# Autodesk Inventor assembly: BATTERY ASSEMBLY
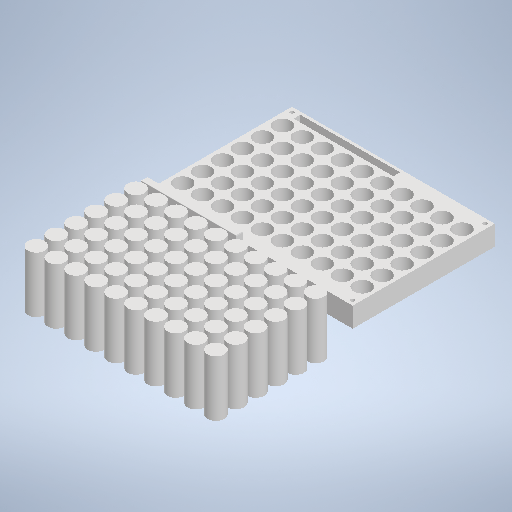
[picture p0: Inventor's stored thumbnail of the model, 512x512]
Saved by Autodesk Inventor 2025.2 (Build 292293000, 293)
## iProperties
Created: 2025-03-22
Part Number: BATTERY ASSEMBLY
Document SubType Name: Assembly
Designer: Mathias
Author: Mathias
## Documents named in this file (4)
- C:\Users\Mathias\Desktop\Projekt Olkassa\Autodesk-inventor-filesharing\BATTERY ASSEMBLY.iam
- C:\Users\Mathias\Desktop\Projekt Olkassa\Autodesk-inventor-filesharing\21700.ipt
- C:\Users\Mathias\Desktop\Projekt Olkassa\Autodesk-inventor-filesharing\BMS.ipt
- C:\Users\Mathias\Desktop\Projekt Olkassa\Autodesk-inventor-filesharing\Battery Holder pt1.ipt
## Components (62 placed, 3 different names)
1. BMS:1
2. Battery Holder pt1:1
3. 21700:1
4. 21700:2
5. 21700:3
6. 21700:4
7. 21700:5
8. 21700:6
9. 21700:7
10. 21700:8
11. 21700:9
12. 21700:10
13. 21700:11
14. 21700:12
15. 21700:13
16. 21700:14
17. 21700:15
18. 21700:16
19. 21700:17
20. 21700:18
21. 21700:19
22. 21700:20
23. 21700:21
24. 21700:22
25. 21700:23
26. 21700:24
27. 21700:25
28. 21700:26
29. 21700:27
30. 21700:28
31. 21700:29
32. 21700:30
33. 21700:31
34. 21700:32
35. 21700:33
36. 21700:34
37. 21700:35
38. 21700:36
39. 21700:37
40. 21700:38
41. 21700:39
42. 21700:40
43. 21700:41
44. 21700:42
45. 21700:43
46. 21700:44
47. 21700:45
48. 21700:46
49. 21700:47
50. 21700:48
51. 21700:49
52. 21700:50
53. 21700:51
54. 21700:52
55. 21700:53
56. 21700:54
57. 21700:55
58. 21700:56
59. 21700:57
60. 21700:58
61. 21700:59
62. 21700:60
## Component patterns: (60 elements, first: 21700:1)
